# Autodesk Inventor assembly: 前底盘组
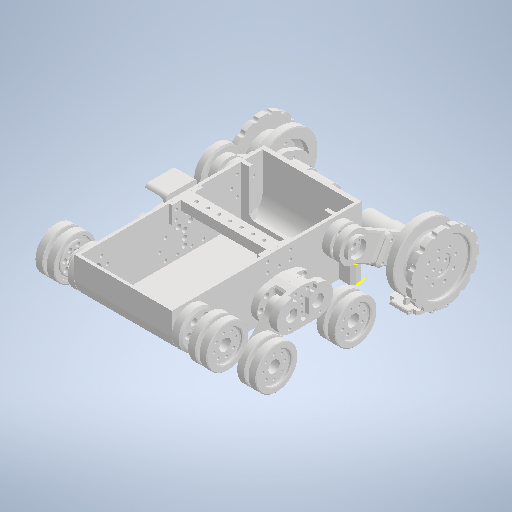
[picture p0: Inventor's stored thumbnail of the model, 512x512]
Saved by Autodesk Inventor 2025.1 (Build 291241000, 241)
## iProperties
Created: 2025-08-27
Part Number: 前底盘组
Document SubType Name: Assembly
Designer: Piw
Author: Piw
## Documents named in this file (17)
- C:\Users\22982\Desktop\急急急\Classis\前底盘组.iam
- C:\Users\22982\Desktop\急急急\Classis\车架.ipt
- C:\Users\22982\Desktop\急急急\Classis\悬架.iam
- C:\Users\22982\Desktop\急急急\Classis\导轮架.ipt
- C:\Users\22982\Desktop\急急急\Classis\内轮.ipt
- C:\Users\22982\Desktop\急急急\Classis\外轮.ipt
- C:\Users\22982\Desktop\急急急\Classis\加强梁.ipt
- C:\Users\22982\Desktop\急急急\Classis\链轮摇臂座.ipt
- C:\Users\22982\Desktop\急急急\Classis\链轮摇臂.ipt
- C:\Users\22982\Desktop\急急急\Classis\JGB37-520.ipt
- C:\Users\22982\Desktop\急急急\Classis\驱动轮法兰.ipt
- C:\Users\22982\Desktop\急急急\Classis\主动轮.ipt
- C:\Users\22982\Desktop\急急急\Classis\主动外轮.ipt
- C:\Users\22982\Desktop\急急急\Classis\履带片.ipt
- C:\Users\22982\Desktop\急急急\Classis\.stp\land.ipt
- C:\Users\22982\Desktop\急急急\Classis\.stp\托带轮.ipt
- C:\Users\22982\Desktop\急急急\Classis\.stp\拖带架.ipt
## Components (27 placed, 16 different names)
1. 车架:1 — 配合:1, 配合:2, 配合:3, 配合:4, 配合:5, 配合:6, 配合:7, 配合:8, 配合:11, 配合:15, 配合:16, 配合:17, 配合:21, 配合:22, 配合:23, 配合:25, 配合:26, 配合:27, 配合:38, 配合:39, 配合:40, 表面齐平:5
2. 悬架:1 [sub-assembly] — 配合:1, 配合:2, 配合:6, 相切:1, 相切:2
3. 悬架:2 [sub-assembly] — 配合:3, 配合:4, 配合:5
4. 导轮架:1 — 配合:7, 配合:8, 配合:11, 旋转:1
5. 内轮:1 — 旋转:1
6. 外轮:1
7. 导轮架:2 — 配合:15, 配合:16, 配合:17, 旋转:2
8. 内轮:2 — 旋转:2
9. 外轮:2
10. 加强梁:1 — 配合:21, 配合:22, 配合:23
11. 链轮摇臂座:1 — 配合:25, 配合:26, 配合:27, 旋转:3
12. 链轮摇臂:1 — 旋转:3, 配合:28, 配合:29, 配合:30
13. JGB37-520:1 — 配合:28, 配合:29, 配合:30, 表面齐平:1, 配合:31
14. 驱动轮法兰:1 — 表面齐平:1, 配合:31, 配合:32, 配合:33, 配合:34
15. 主动轮:1 — 配合:32, 配合:33, 配合:34, 配合:35, 配合:36, 配合:37, 配合:52, 相切:3
16. 主动外轮:1 — 配合:35, 配合:36, 配合:37, 配合:51
17. 链轮摇臂座:2 — 配合:38, 配合:39, 配合:40, 旋转:4
18. 链轮摇臂:2 — 旋转:4, 配合:41, 配合:42, 配合:43, 表面齐平:4
19. JGB37-520:2 — 配合:41, 配合:42, 配合:43, 表面齐平:2, 配合:44
20. 驱动轮法兰:2 — 表面齐平:2, 配合:44, 配合:45, 配合:46, 配合:47
21. 主动轮:2 — 配合:45, 配合:46, 配合:47, 配合:48, 配合:49, 配合:50
22. 主动外轮:2 — 配合:48, 配合:49, 配合:50
23. 履带片:1 — 配合:51, 配合:52, 配合:53, 表面齐平:3
24. 履带片:2 — 配合:53, 表面齐平:3
25. land:1 — 相切:1, 相切:2, 相切:3
26. 托带轮:1 — 表面齐平:4
27. 拖带架:1 — 表面齐平:5
## Relationships (62: Mate 50, Flush 5, RevoluteJoint 4, Tangent 3)
- 配合:1 [Mate]: 车架:1 ↔ 悬架:1
- 配合:2 [Mate]: 车架:1 ↔ 悬架:1
- 配合:3 [Mate]: 车架:1 ↔ 悬架:2
- 配合:4 [Mate]: 车架:1 ↔ 悬架:2
- 配合:5 [Mate]: 车架:1 ↔ 悬架:2
- 配合:6 [Mate]: 车架:1 ↔ 悬架:1
- 配合:7 [Mate]: 车架:1 ↔ 导轮架:1
- 配合:8 [Mate]: 车架:1 ↔ 导轮架:1
- 配合:11 [Mate]: 车架:1 ↔ 导轮架:1
- [Mate]: 内轮:1 ↔ 外轮:1
- [Mate]: 内轮:1 ↔ 外轮:1
- [Mate]: 内轮:1 ↔ 外轮:1
- 旋转:1 [RevoluteJoint]: 导轮架:1 ↔ 内轮:1
- 配合:15 [Mate]: 车架:1 ↔ 导轮架:2
- 配合:16 [Mate]: 车架:1 ↔ 导轮架:2
- 配合:17 [Mate]: 车架:1 ↔ 导轮架:2
- [Mate]: 内轮:2 ↔ 外轮:2
- [Mate]: 内轮:2 ↔ 外轮:2
- [Mate]: 内轮:2 ↔ 外轮:2
- 旋转:2 [RevoluteJoint]: 导轮架:2 ↔ 内轮:2
- 配合:21 [Mate]: 车架:1 ↔ 加强梁:1
- 配合:22 [Mate]: 车架:1 ↔ 加强梁:1
- 配合:23 [Mate]: 车架:1 ↔ 加强梁:1
- 配合:25 [Mate]: 车架:1 ↔ 链轮摇臂座:1
- 配合:26 [Mate]: 车架:1 ↔ 链轮摇臂座:1
- 配合:27 [Mate]: 车架:1 ↔ 链轮摇臂座:1
- 旋转:3 [RevoluteJoint] (-7 mm): 链轮摇臂座:1 ↔ 链轮摇臂:1
- 配合:28 [Mate]: 链轮摇臂:1 ↔ JGB37-520:1
- 配合:29 [Mate]: 链轮摇臂:1 ↔ JGB37-520:1
- 配合:30 [Mate]: 链轮摇臂:1 ↔ JGB37-520:1
- 表面齐平:1 [Flush]: JGB37-520:1 ↔ 驱动轮法兰:1
- 配合:31 [Mate]: JGB37-520:1 ↔ 驱动轮法兰:1
- 配合:32 [Mate]: 驱动轮法兰:1 ↔ 主动轮:1
- 配合:33 [Mate]: 驱动轮法兰:1 ↔ 主动轮:1
- 配合:34 [Mate]: 驱动轮法兰:1 ↔ 主动轮:1
- 配合:35 [Mate]: 主动轮:1 ↔ 主动外轮:1
- 配合:36 [Mate]: 主动轮:1 ↔ 主动外轮:1
- 配合:37 [Mate]: 主动轮:1 ↔ 主动外轮:1
- 配合:38 [Mate]: 车架:1 ↔ 链轮摇臂座:2
- 配合:39 [Mate]: 车架:1 ↔ 链轮摇臂座:2
- 配合:40 [Mate]: 车架:1 ↔ 链轮摇臂座:2
- 旋转:4 [RevoluteJoint]: 链轮摇臂座:2 ↔ 链轮摇臂:2
- 配合:41 [Mate]: 链轮摇臂:2 ↔ JGB37-520:2
- 配合:42 [Mate]: 链轮摇臂:2 ↔ JGB37-520:2
- 配合:43 [Mate]: 链轮摇臂:2 ↔ JGB37-520:2
- 表面齐平:2 [Flush]: JGB37-520:2 ↔ 驱动轮法兰:2
- 配合:44 [Mate]: JGB37-520:2 ↔ 驱动轮法兰:2
- 配合:45 [Mate]: 驱动轮法兰:2 ↔ 主动轮:2
- 配合:46 [Mate]: 驱动轮法兰:2 ↔ 主动轮:2
- 配合:47 [Mate]: 驱动轮法兰:2 ↔ 主动轮:2
- 配合:48 [Mate]: 主动轮:2 ↔ 主动外轮:2
- 配合:49 [Mate]: 主动轮:2 ↔ 主动外轮:2
- 配合:50 [Mate]: 主动轮:2 ↔ 主动外轮:2
- 配合:51 [Mate]: 主动外轮:1 ↔ 履带片:1
- 配合:52 [Mate] (1 mm): 主动轮:1 ↔ 履带片:1
- 配合:53 [Mate]: 履带片:1 ↔ 履带片:2
- 表面齐平:3 [Flush]: 履带片:1 ↔ 履带片:2
- 相切:1 [Tangent]: 悬架:1 ↔ land:1
- 相切:2 [Tangent]: 悬架:1 ↔ land:1
- 相切:3 [Tangent]: 主动轮:1 ↔ land:1
- 表面齐平:4 [Flush]: 链轮摇臂:2 ↔ 托带轮:1
- 表面齐平:5 [Flush]: 车架:1 ↔ 拖带架:1
## Named parameters: d28_d22 = 0 mm, d29_d23 = 0 mm, d30_d28_d22 = 0 mm, d31_d29_d23 = 0 mm, d33_d32 = 0 mm
